# Autodesk Inventor assembly: licht_150_MIR
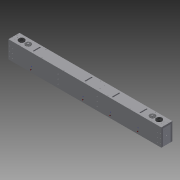
[picture p0: Inventor's stored thumbnail of the model, 180x180]
Saved by Autodesk Inventor 2015 (Build 190159000, 159)
## iProperties
Created: 2018-02-17
Part Number: licht_150_MIR
Document SubType Name: Assembly
Designer: wepet
Author: wepet
## Documents named in this file (13)
- C:\workspace\robosax\licht\Alles\licht_150_MIR.iam
- C:\workspace\robosax\licht\Alles\licht_150_back_MIR.ipt
- C:\workspace\robosax\licht\Alles\licht_150_front_MIR.ipt
- C:\workspace\robosax\licht\Alles\licht_150_top_MIR.ipt
- C:\workspace\robosax\licht\Alles\licht_150_side_middle_MIR.ipt
- C:\workspace\robosax\licht\Zusatzelemente\licht_led_blau_MIR.ipt
- C:\workspace\robosax\licht\Zusatzelemente\licht_taster_MIR.ipt
- C:\workspace\robosax\licht\Zusatzelemente\anschluss_strom_MIR.ipt
- C:\workspace\robosax\licht\Zusatzelemente\anschluss_daten_MIR.iam
- C:\workspace\robosax\licht\Alles\licht_150_side_right_MIR.ipt
- C:\workspace\robosax\licht\Alles\licht_150_side_left_MIR.ipt
- C:\workspace\robosax\licht\Alles\licht_150_support_right_MIR.ipt
- C:\workspace\robosax\licht\Alles\licht_150_support_left_MIR.ipt
## Components (20 placed, 12 different names)
1. licht_150_back_MIR:1 — Fluchtend:4, Fluchtend:3, Fluchtend:5, Passend:9, Fluchtend:13
2. licht_150_front_MIR:1 — Fluchtend:4, Fluchtend:3, Passend:3, Passend:2, Passend:1, Fluchtend:2, Fluchtend:1, Passend:4, Passend:36, Einfügen:4, Einfügen:3, Einfügen:1, Einfügen:2, Einfügen:5, Einfügen:6, Einfügen:7, Einfügen:8, Fluchtend:12, Passend:37, Passend:39, Passend:42, Passend:45
3. licht_150_top_MIR:1 — Fluchtend:5, Fluchtend:2, Fluchtend:1, Passend:4, Passend:8, Passend:26, Passend:31, Passend:30, Passend:29, Passend:28, Passend:27, Passend:34, Passend:33, Passend:32, Passend:38, Passend:40, Passend:41, Passend:44, Drehbar:1
4. licht_150_side_middle_MIR:1 — Passend:36, Passend:9, Passend:8
5. licht_led_blau_MIR:1 — Einfügen:4
6. licht_led_blau_MIR:2 — Einfügen:3
7. licht_led_blau_MIR:3 — Einfügen:1
8. licht_led_blau_MIR:4 — Einfügen:2
9. licht_taster_MIR:1 — Einfügen:5
10. licht_taster_MIR:2 — Einfügen:6
11. licht_taster_MIR:3 — Einfügen:7
12. licht_taster_MIR:4 — Einfügen:8
13. anschluss_strom_MIR:1 — Passend:26, Drehbar:1
14. anschluss_strom_MIR:2 — Passend:31, Passend:30
15. anschluss_daten_MIR:1 [sub-assembly] — Passend:29, Passend:28, Passend:27
16. anschluss_daten_MIR:2 [sub-assembly] — Passend:34, Passend:33, Passend:32
17. licht_150_side_right_MIR:1 — Passend:38, Fluchtend:12, Passend:37, Passend:43
18. licht_150_side_left_MIR:1 — Fluchtend:13, Passend:40, Passend:39, Passend:46
19. licht_150_support_right_MIR:1 — Passend:43, Passend:42, Passend:41
20. licht_150_support_left_MIR:1 — Passend:46, Passend:45, Passend:44
## Relationships (42: Mate 25, Flush 8, Insert 8, RevoluteJoint 1)
- Fluchtend:4 [Flush]: licht_150_back_MIR:1 ↔ licht_150_front_MIR:1
- Fluchtend:3 [Flush]: licht_150_back_MIR:1 ↔ licht_150_front_MIR:1
- Passend:3 [Mate]: licht_150_front_MIR:1
- Passend:2 [Flush]: licht_150_front_MIR:1
- Passend:1 [Mate]: licht_150_front_MIR:1
- Fluchtend:5 [Flush]: licht_150_back_MIR:1 ↔ licht_150_top_MIR:1
- Fluchtend:2 [Flush]: licht_150_front_MIR:1 ↔ licht_150_top_MIR:1
- Fluchtend:1 [Flush]: licht_150_front_MIR:1 ↔ licht_150_top_MIR:1
- Passend:4 [Mate]: licht_150_front_MIR:1 ↔ licht_150_top_MIR:1
- Passend:36 [Mate]: licht_150_front_MIR:1 ↔ licht_150_side_middle_MIR:1
- Passend:9 [Mate]: licht_150_back_MIR:1 ↔ licht_150_side_middle_MIR:1
- Passend:8 [Mate]: licht_150_top_MIR:1 ↔ licht_150_side_middle_MIR:1
- Einfügen:4 [Insert]: licht_150_front_MIR:1 ↔ licht_led_blau_MIR:1
- Einfügen:3 [Insert]: licht_150_front_MIR:1 ↔ licht_led_blau_MIR:2
- Einfügen:1 [Insert] (-5 mm): licht_150_front_MIR:1 ↔ licht_led_blau_MIR:3
- Einfügen:2 [Insert] (-5 mm): licht_150_front_MIR:1 ↔ licht_led_blau_MIR:4
- Einfügen:5 [Insert] (5 mm): licht_150_front_MIR:1 ↔ licht_taster_MIR:1
- Einfügen:6 [Insert] (5 mm): licht_150_front_MIR:1 ↔ licht_taster_MIR:2
- Einfügen:7 [Insert] (5 mm): licht_150_front_MIR:1 ↔ licht_taster_MIR:3
- Einfügen:8 [Insert] (5 mm): licht_150_front_MIR:1 ↔ licht_taster_MIR:4
- Passend:26 [Mate]: licht_150_top_MIR:1 ↔ anschluss_strom_MIR:1
- Passend:31 [Mate]: licht_150_top_MIR:1 ↔ anschluss_strom_MIR:2
- Passend:30 [Mate]: licht_150_top_MIR:1 ↔ anschluss_strom_MIR:2
- Passend:29 [Mate]: licht_150_top_MIR:1 ↔ anschluss_daten_MIR:1
- Passend:28 [Mate]: licht_150_top_MIR:1 ↔ anschluss_daten_MIR:1
- Passend:27 [Mate]: licht_150_top_MIR:1 ↔ anschluss_daten_MIR:1
- Passend:34 [Mate]: licht_150_top_MIR:1 ↔ anschluss_daten_MIR:2
- Passend:33 [Mate]: licht_150_top_MIR:1 ↔ anschluss_daten_MIR:2
- Passend:32 [Mate]: licht_150_top_MIR:1 ↔ anschluss_daten_MIR:2
- Passend:38 [Mate]: licht_150_top_MIR:1 ↔ licht_150_side_right_MIR:1
- Fluchtend:12 [Flush]: licht_150_front_MIR:1 ↔ licht_150_side_right_MIR:1
- Passend:37 [Mate]: licht_150_front_MIR:1 ↔ licht_150_side_right_MIR:1
- Fluchtend:13 [Flush]: licht_150_back_MIR:1 ↔ licht_150_side_left_MIR:1
- Passend:40 [Mate]: licht_150_top_MIR:1 ↔ licht_150_side_left_MIR:1
- Passend:39 [Mate]: licht_150_front_MIR:1 ↔ licht_150_side_left_MIR:1
- Passend:43 [Mate]: licht_150_side_right_MIR:1 ↔ licht_150_support_right_MIR:1
- Passend:42 [Mate]: licht_150_front_MIR:1 ↔ licht_150_support_right_MIR:1
- Passend:41 [Mate]: licht_150_top_MIR:1 ↔ licht_150_support_right_MIR:1
- Passend:46 [Mate]: licht_150_side_left_MIR:1 ↔ licht_150_support_left_MIR:1
- Passend:45 [Mate]: licht_150_front_MIR:1 ↔ licht_150_support_left_MIR:1
- Passend:44 [Mate]: licht_150_top_MIR:1 ↔ licht_150_support_left_MIR:1
- Drehbar:1 [RevoluteJoint] (7 mm): licht_150_top_MIR:1 ↔ anschluss_strom_MIR:1
